# Autodesk Inventor assembly: support_frameAssembly
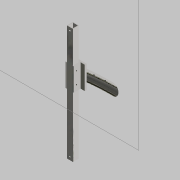
[picture p0: Inventor's stored thumbnail of the model, 180x180]
Saved by Autodesk Inventor 2021 (Build 250183000, 183)
## iProperties
Created: 2021-05-25
Part Number: support_frameAssembly
Document SubType Name: Assembly
Designer: Watchdog
Author: Watchdog
## Documents named in this file (3)
- C:\Users\Watchdog\OneDrive - Flinders\Advn Mech Design Shared\6_Development\2_Design\inventor\support\support_frameAssembly.iam
- C:\Users\Watchdog\OneDrive - Flinders\Advn Mech Design Shared\6_Development\2_Design\inventor\support\support_frame_x.ipt
- C:\Users\Watchdog\OneDrive - Flinders\Advn Mech Design Shared\6_Development\2_Design\inventor\support\support_basePart.ipt
## Components (2 placed, 2 different names)
1. support_frame_x:1 — Flush:1, Mate:1, Flush:2, Mate:2, Mate:3, Mate:4
2. support_basePart:1 — Mate:2, Mate:3, Mate:4
## Relationships (6: Mate 4, Flush 2)
- Flush:1: support_frame_x:1
- Mate:1: support_frame_x:1
- Flush:2: support_frame_x:1
- Mate:2: support_frame_x:1 ↔ support_basePart:1
- Mate:3: support_frame_x:1 ↔ support_basePart:1
- Mate:4: support_frame_x:1 ↔ support_basePart:1
